# Autodesk Inventor assembly: Fuellsimulation_V1
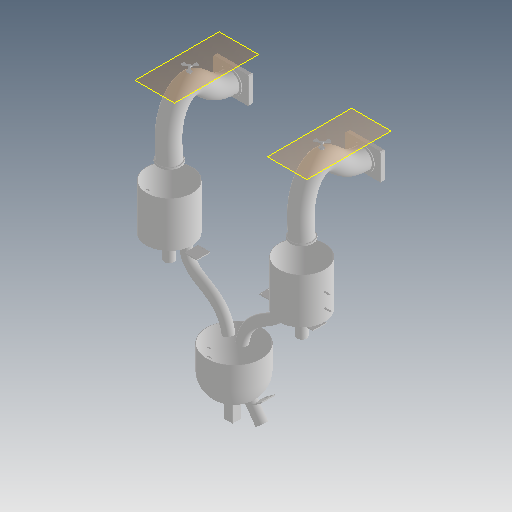
[picture p0: Inventor's stored thumbnail of the model, 512x512]
Saved by Autodesk Inventor 2020 (Build 240168000, 168)
## iProperties
Created: 2020-04-06
Part Number: Fuellsimulation_V1
Document SubType Name: Assembly
Designer: franz
Author: franz
## Documents named in this file (11)
- E:\Privat\Projekte\SPS_Training\Unity_SPS_Simulation\Unity_SPS_Schrittkette\CAD\Fuellsimulation_V1\Fuellsimulation_V1.iam
- E:\Privat\Projekte\SPS_Training\Unity_SPS_Simulation\Unity_SPS_Schrittkette\CAD\Fuellsimulation_V1\Tank_1.ipt
- E:\Privat\Projekte\SPS_Training\Unity_SPS_Simulation\Unity_SPS_Schrittkette\CAD\Fuellsimulation_V1\Rohr_1.ipt
- E:\Privat\Projekte\SPS_Training\Unity_SPS_Simulation\Unity_SPS_Schrittkette\CAD\Fuellsimulation_V1\Tank_3.ipt
- E:\Privat\Projekte\SPS_Training\Unity_SPS_Simulation\Unity_SPS_Schrittkette\CAD\Fuellsimulation_V1\Rohr_2.ipt
- E:\Privat\Projekte\SPS_Training\Unity_SPS_Simulation\Unity_SPS_Schrittkette\CAD\Fuellsimulation_V1\Ruehrwerk.ipt
- E:\Privat\Projekte\SPS_Training\Unity_SPS_Simulation\Unity_SPS_Schrittkette\CAD\Fuellsimulation_V1\Motor.ipt
- E:\Privat\Projekte\SPS_Training\Unity_SPS_Simulation\Unity_SPS_Schrittkette\CAD\Fuellsimulation_V1\Ventil.ipt
- E:\Privat\Projekte\SPS_Training\Unity_SPS_Simulation\Unity_SPS_Schrittkette\CAD\Fuellsimulation_V1\Heizwendel.ipt
- E:\Privat\Projekte\SPS_Training\Unity_SPS_Simulation\Unity_SPS_Schrittkette\CAD\Fuellsimulation_V1\Sensor.ipt
- E:\Privat\Projekte\SPS_Training\Unity_SPS_Simulation\Unity_SPS_Schrittkette\CAD\Fuellsimulation_V1\Rohr_3.ipt
## Components (26 placed, 10 different names)
1. Tank_1:1 — Starr:1, Fluchtend:1, Passend:1, Fluchtend:2, Starr:3, Passend:2
2. Tank_1:2 — Starr:2, Fluchtend:1, Passend:1, Starr:4, Passend:3
3. Rohr_1:1 — Starr:1
4. Rohr_1:2 — Starr:2
5. Tank_3:1 — Fluchtend:2, Starr:5
6. Rohr_2:1 — Starr:3
7. Rohr_2:2 — Starr:5
8. Rohr_2:3 — Starr:4
9. Ruehrwerk:1 — Starr:6
10. Motor:1 — Starr:6
11. Ventil:1
12. Heizwendel:1
13. Sensor:1
14. Rohr_3:1 — Fluchtend:3, Fluchtend:4, Passend:3
15. Heizwendel:2
16. Sensor:2
17. Sensor:3
18. Sensor:4
19. Sensor:5
20. Sensor:6
21. Sensor:7
22. Rohr_3:2 — Fluchtend:3, Fluchtend:4, Passend:2
23. Ventil:2
24. Ventil:3
25. Ventil:4
26. Ventil:5
## Relationships (13: WeldJoint 6, Flush 4, Mate 3)
- Starr:1 [WeldJoint]: Tank_1:1 ↔ Rohr_1:1
- Starr:2 [WeldJoint]: Tank_1:2 ↔ Rohr_1:2
- Fluchtend:1 [Flush]: Tank_1:1 ↔ Tank_1:2
- Passend:1 [Mate]: Tank_1:1 ↔ Tank_1:2
- Fluchtend:2 [Flush]: Tank_1:1 ↔ Tank_3:1
- Starr:3 [WeldJoint]: Tank_1:1 ↔ Rohr_2:1
- Starr:4 [WeldJoint]: Tank_1:2 ↔ Rohr_2:3
- Starr:5 [WeldJoint]: Tank_3:1 ↔ Rohr_2:2
- Starr:6 [WeldJoint]: Ruehrwerk:1 ↔ Motor:1
- Fluchtend:3 [Flush]: Rohr_3:1 ↔ Rohr_3:2
- Fluchtend:4 [Flush]: Rohr_3:1 ↔ Rohr_3:2
- Passend:2 [Mate]: Tank_1:1 ↔ Rohr_3:2
- Passend:3 [Mate]: Tank_1:2 ↔ Rohr_3:1
